# Autodesk Inventor assembly: Assembly
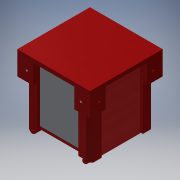
[picture p0: Inventor's stored thumbnail of the model, 180x180]
Saved by Autodesk Inventor 2018 (Build 220112000, 112)
## iProperties
Created: 2019-10-03
Part Number: Assembly
Document SubType Name: Assembly
Designer: Ivan
Author: Ivan
## Documents named in this file (5)
- C:\Users\Ivan\Documents\GitHub\Sensor-de-Vibraciones\Faraday\Assembly.iam
- C:\Users\Ivan\Documents\GitHub\Sensor-de-Vibraciones\Faraday\Bottom.ipt
- C:\Users\Ivan\Documents\GitHub\Sensor-de-Vibraciones\Faraday\TopBox.ipt
- C:\Users\Ivan\Documents\GitHub\Sensor-de-Vibraciones\Faraday\Flat52.ipt
- C:\Users\Ivan\Documents\GitHub\Sensor-de-Vibraciones\Faraday\Flat60.ipt
## Components (4 placed, 4 different names)
1. Bottom:1 — Insert:1, Insert:2, Flush:1, Mate:5
2. TopBox:1 — Insert:1, Insert:2, Mate:1, Mate:2, Mate:3, Mate:4, Mate:6
3. Flat52:1 — Mate:1, Mate:2, Mate:3
4. Flat60:1 — Mate:4, Mate:5, Mate:6
## Relationships (9: Mate 6, Insert 2, Flush 1)
- Insert:1: Bottom:1 ↔ TopBox:1
- Insert:2: Bottom:1 ↔ TopBox:1
- Flush:1: Bottom:1
- Mate:1: TopBox:1 ↔ Flat52:1
- Mate:2: TopBox:1 ↔ Flat52:1
- Mate:3: TopBox:1 ↔ Flat52:1
- Mate:4: TopBox:1 ↔ Flat60:1
- Mate:5: Bottom:1 ↔ Flat60:1
- Mate:6: TopBox:1 ↔ Flat60:1
